# Autodesk Inventor assembly: West_Test_Structure
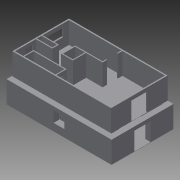
[picture p0: Inventor's stored thumbnail of the model, 180x180]
Saved by Autodesk Inventor 2013 SP2 (Build 170200200, 200)
## iProperties
Created: 2014-07-16
Part Number: West_Test_Structure
Document SubType Name: Assembly
Designer: jmw3
Author: jmw3
## Documents named in this file (3)
- C:\Users\jmw3\Documents\Structure Drawings\DelCo_Drawings\Inventor Files\Models\West_Test_Structure.iam
- C:\Users\jmw3\Documents\Structure Drawings\DelCo_Drawings\Inventor Files\Models\West_Test_Structure_1st_Floor.ipt
- C:\Users\jmw3\Documents\Structure Drawings\DelCo_Drawings\Inventor Files\Models\West_Test_Structure_2nd_Floor.ipt
## Components (2 placed, 2 different names)
1. West_Test_Structure_1st_Floor:1 — Flush:1, Mate:1, Flush:2
2. West_Test_Structure_2nd_Floor:1 — Flush:1, Mate:1, Flush:2, Flush:3, Flush:4
## Relationships (5: Flush 4, Mate 1)
- Flush:1 (304.8 mm): West_Test_Structure_1st_Floor:1 ↔ West_Test_Structure_2nd_Floor:1
- Mate:1 (298.45 mm): West_Test_Structure_1st_Floor:1 ↔ West_Test_Structure_2nd_Floor:1
- Flush:2 (355.6 mm): West_Test_Structure_1st_Floor:1 ↔ West_Test_Structure_2nd_Floor:1
- Flush:3 (-304.8 mm): West_Test_Structure_2nd_Floor:1
- Flush:4 (-5461 mm): West_Test_Structure_2nd_Floor:1
